# Autodesk Inventor assembly: mg996r 3mm left leg
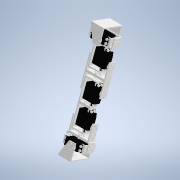
[picture p0: Inventor's stored thumbnail of the model, 180x180]
Saved by Autodesk Inventor 2021.4 (Build 254397000, 397)
## iProperties
Created: 2022-07-09
Part Number: mg996r 3mm left leg
Document SubType Name: Assembly
Designer: isamu
Author: isamu
## Documents named in this file (6)
- D:\personal_projects\robot\inventor\2021\mg996r 3mm left leg.iam
- D:\personal_projects\robot\inventor\2021\base mg996r 3mm centered left.iam
- D:\personal_projects\robot\inventor\2021\mg996r 3mm frame middle leg.iam
- D:\personal_projects\robot\exports\screws\m4 nuts.ipt
- D:\personal_projects\robot\inventor\2021\base mg996r 3mm left foot.iam
- D:\personal_projects\robot\exports\screws\m3 nuts.ipt
## Components (13 placed, 5 different names)
1. base mg996r 3mm centered left:1 [sub-assembly] — Mate:1, Mate:2, Mate:3, Insert:1, Insert:2, Insert:3, Insert:4, Insert:5
2. mg996r 3mm frame middle leg:1 [sub-assembly] — Mate:1, Mate:2, Mate:3, Mate:4, Mate:5, Mate:6
3. m4 nuts:1 — Insert:2
4. m4 nuts:2 — Insert:1
5. m4 nuts:3 — Insert:4
6. m4 nuts:4 — Insert:5
7. m4 nuts:5 — Insert:3
8. base mg996r 3mm left foot:1 [sub-assembly] — Mate:4, Mate:5, Mate:6, Insert:6, Insert:7, Insert:8, Insert:9, Insert:10
9. m3 nuts:1 — Insert:8
10. m3 nuts:2 — Insert:6
11. m3 nuts:3 — Insert:10
12. m3 nuts:4 — Insert:7
13. m3 nuts:5 — Insert:9
## Relationships (16: Insert 10, Mate 6)
- Mate:1: base mg996r 3mm centered left:1 ↔ mg996r 3mm frame middle leg:1
- Mate:2: base mg996r 3mm centered left:1 ↔ mg996r 3mm frame middle leg:1
- Mate:3: base mg996r 3mm centered left:1 ↔ mg996r 3mm frame middle leg:1
- Insert:1: base mg996r 3mm centered left:1 ↔ m4 nuts:2
- Insert:2: base mg996r 3mm centered left:1 ↔ m4 nuts:1
- Insert:3: base mg996r 3mm centered left:1 ↔ m4 nuts:5
- Insert:4: base mg996r 3mm centered left:1 ↔ m4 nuts:3
- Insert:5: base mg996r 3mm centered left:1 ↔ m4 nuts:4
- Mate:4: mg996r 3mm frame middle leg:1 ↔ base mg996r 3mm left foot:1
- Mate:5: mg996r 3mm frame middle leg:1 ↔ base mg996r 3mm left foot:1
- Mate:6: mg996r 3mm frame middle leg:1 ↔ base mg996r 3mm left foot:1
- Insert:6: base mg996r 3mm left foot:1 ↔ m3 nuts:2
- Insert:7: base mg996r 3mm left foot:1 ↔ m3 nuts:4
- Insert:8: base mg996r 3mm left foot:1 ↔ m3 nuts:1
- Insert:9: base mg996r 3mm left foot:1 ↔ m3 nuts:5
- Insert:10: base mg996r 3mm left foot:1 ↔ m3 nuts:3
